# Autodesk Inventor assembly: 742 2.1 Blocker
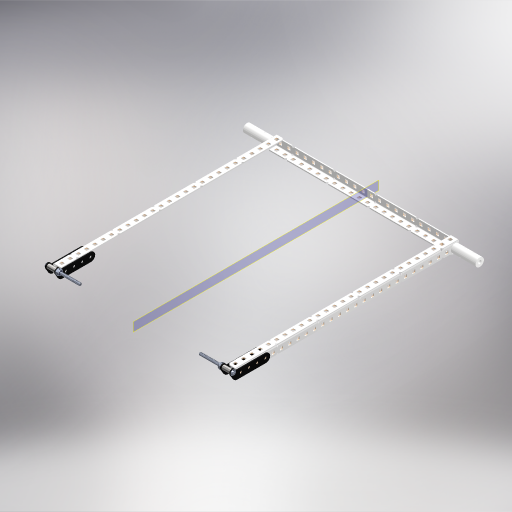
[picture p0: Inventor's stored thumbnail of the model, 512x512]
Saved by Autodesk Inventor 2024 (Build 280153000, 153)
## iProperties
Created: 2023-10-21
Part Number: 742 2.1 Blocker
Document SubType Name: Assembly
Designer: aaron
Author: aaron
## Documents named in this file (10)
- C:\Users\aaron\Documents\Inventor\TritonRobotics\library\Subsystems\742 2.1 Blocker.iam
- C:\Users\aaron\Documents\Inventor\TritonRobotics\library\VEX Library\Structure\C-Channels\Aluminum 1x1 from VEX\1x1x27 Aluminum Angle.ipt
- C:\Users\aaron\Documents\Inventor\TritonRobotics\library\Stock Material\Plates New\Blocker Gusset.ipt
- C:\Users\aaron\Documents\Inventor\TritonRobotics\library\VEX Library\Structure\C-Channels\Aluminum 1x1 from VEX\1x1x22 Aluminum Angle.ipt
- C:\Users\aaron\Documents\Inventor\TritonRobotics\library\VEX Library\Motion\Spacers\Spacer (Nylon), .500 OD\0.5 in.ipt
- C:\Users\aaron\Documents\Inventor\TritonRobotics\library\VEX Library\Motion\Spacers\Spacer (Nylon), .500 OD.ipt
- C:\Users\aaron\Documents\Inventor\TritonRobotics\library\VEX Library\Structure\Hardware\Screw Steel - Star\Screw 8-32 Steel 2.000.ipt
- C:\Users\aaron\Documents\Inventor\TritonRobotics\library\VEX Library\Structure\Hardware\Screw Steel - Star.ipt
- C:\Users\aaron\Documents\Inventor\TritonRobotics\library\VEX Library\Structure\Hardware\Nut Thin Nylock.ipt
- C:\Users\aaron\Documents\Inventor\TritonRobotics\library\VEX Library\Structure\Metal Spacers\0.25 1-2 od.ipt
## Components (21 placed, 7 different names)
1. 1x1x27 Aluminum Angle:1 — Mate:1, Mate:2, Mate:9, Mate:10, Mate:11, Mate:13, Mate:15, Mate:28, Mate:29, Symmetry:1
2. 1x1x27 Aluminum Angle:2 — Mate:1, Mate:2, Mate:3, Mate:4, Mate:5, Mate:7, Mate:16, Mate:17, Mate:22, Mate:23, Symmetry:1
3. Blocker Gusset:1 — Mate:3, Mate:4, Mate:5, Mate:6, Mate:8, Mate:32, Mate:33, Mate:44
4. Blocker Gusset:2 — Mate:6, Mate:7, Mate:8, Mate:35
5. Blocker Gusset:3 — Mate:9, Mate:10, Mate:11, Mate:12, Mate:14, Mate:30, Mate:31
6. Blocker Gusset:4 — Mate:12, Mate:13, Mate:14, Mate:37, Mate:40
7. 1x1x22 Aluminum Angle:2 — Mate:15, Mate:16, Mate:17
8. 0.5 in:1 — Mate:18, Mate:19, Mate:23
9. 0.5 in:2 — Mate:18, Mate:19, Mate:20, Mate:21
10. 0.5 in:3 — Mate:20, Mate:21, Mate:22
11. 0.5 in:4 — Mate:28
12. 0.5 in:5 — Mate:29
13. 0.5 in:6
14. Screw 8-32 Steel 2.000:1 — Mate:32, Mate:33, Mate:34, Mate:45
15. Screw 8-32 Steel 2.000:2 — Mate:30, Mate:31, Mate:36, Mate:41
16. Nut Thin Nylock:1 — Mate:34, Mate:35
17. Nut Thin Nylock:2 — Mate:36, Mate:37
18. 0.25 1-2 od:2 — Mate:38, Mate:39, Mate:40, Mate:41
19. 0.25 1-2 od:3 — Mate:38, Mate:39
20. 0.25 1-2 od:4
21. 0.25 1-2 od:5 — Mate:44, Mate:45
## Relationships (46: Mate 45, Symmetry 1)
- Mate:1: 1x1x27 Aluminum Angle:1 ↔ 1x1x27 Aluminum Angle:2
- Mate:2: 1x1x27 Aluminum Angle:1 ↔ 1x1x27 Aluminum Angle:2
- Mate:3: 1x1x27 Aluminum Angle:2 ↔ Blocker Gusset:1
- Mate:4: 1x1x27 Aluminum Angle:2 ↔ Blocker Gusset:1
- Mate:5: 1x1x27 Aluminum Angle:2 ↔ Blocker Gusset:1
- Mate:6: Blocker Gusset:1 ↔ Blocker Gusset:2
- Mate:7: 1x1x27 Aluminum Angle:2 ↔ Blocker Gusset:2
- Mate:8 (12.7 mm): Blocker Gusset:1 ↔ Blocker Gusset:2
- Mate:9: 1x1x27 Aluminum Angle:1 ↔ Blocker Gusset:3
- Mate:10: 1x1x27 Aluminum Angle:1 ↔ Blocker Gusset:3
- Mate:11: 1x1x27 Aluminum Angle:1 ↔ Blocker Gusset:3
- Mate:12: Blocker Gusset:3 ↔ Blocker Gusset:4
- Mate:13: 1x1x27 Aluminum Angle:1 ↔ Blocker Gusset:4
- Mate:14 (12.7 mm): Blocker Gusset:3 ↔ Blocker Gusset:4
- Mate:15: 1x1x27 Aluminum Angle:1 ↔ 1x1x22 Aluminum Angle:2
- Mate:16: 1x1x27 Aluminum Angle:2 ↔ 1x1x22 Aluminum Angle:2
- Mate:17 (12.7 mm): 1x1x27 Aluminum Angle:2 ↔ 1x1x22 Aluminum Angle:2
- Mate:18: 0.5 in:1 ↔ 0.5 in:2
- Mate:19: 0.5 in:1 ↔ 0.5 in:2
- Mate:20: 0.5 in:2 ↔ 0.5 in:3
- Mate:21: 0.5 in:2 ↔ 0.5 in:3
- Mate:22: 1x1x27 Aluminum Angle:2 ↔ 0.5 in:3
- Mate:23: 1x1x27 Aluminum Angle:2 ↔ 0.5 in:1
- [Mate]: 0.5 in:4 ↔ 0.5 in:5
- [Mate]: 0.5 in:4 ↔ 0.5 in:5
- [Mate]: 0.5 in:5 ↔ 0.5 in:6
- [Mate]: 0.5 in:5 ↔ 0.5 in:6
- Mate:28: 1x1x27 Aluminum Angle:1 ↔ 0.5 in:4
- Mate:29: 1x1x27 Aluminum Angle:1 ↔ 0.5 in:5
- Mate:30: Blocker Gusset:3 ↔ Screw 8-32 Steel 2.000:2
- Mate:31: Blocker Gusset:3 ↔ Screw 8-32 Steel 2.000:2
- Mate:32: Blocker Gusset:1 ↔ Screw 8-32 Steel 2.000:1
- Mate:33: Blocker Gusset:1 ↔ Screw 8-32 Steel 2.000:1
- Mate:34: Screw 8-32 Steel 2.000:1 ↔ Nut Thin Nylock:1
- Mate:35: Blocker Gusset:2 ↔ Nut Thin Nylock:1
- Mate:36: Screw 8-32 Steel 2.000:2 ↔ Nut Thin Nylock:2
- Mate:37: Blocker Gusset:4 ↔ Nut Thin Nylock:2
- Mate:38: 0.25 1-2 od:2 ↔ 0.25 1-2 od:3
- Mate:39: 0.25 1-2 od:2 ↔ 0.25 1-2 od:3
- Mate:40: Blocker Gusset:4 ↔ 0.25 1-2 od:2
- Mate:41: Screw 8-32 Steel 2.000:2 ↔ 0.25 1-2 od:2
- [Mate]: 0.25 1-2 od:4 ↔ 0.25 1-2 od:5
- [Mate]: 0.25 1-2 od:4 ↔ 0.25 1-2 od:5
- Mate:44: Blocker Gusset:1 ↔ 0.25 1-2 od:5
- Mate:45: Screw 8-32 Steel 2.000:1 ↔ 0.25 1-2 od:5
- Symmetry:1: 1x1x27 Aluminum Angle:1 ↔ 1x1x27 Aluminum Angle:2
## Named parameters: d24_d18 = 0 mm, d25_d19 = 0 mm, d26_d20 = 0 mm, d27_d21 = 0 mm, d42_d38 = 0 mm, d43_d39 = 0 mm
